# Autodesk Inventor assembly: Gondola
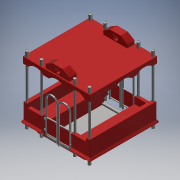
[picture p0: Inventor's stored thumbnail of the model, 180x180]
Saved by Autodesk Inventor 2018 (Build 220112000, 112)
## iProperties
Created: 2018-02-09
Part Number: Gondola
Document SubType Name: Assembly
Designer: Joey
Author: Joey
## Documents named in this file (13)
- M:\TPS\9th Grade\CADD 2017-2018\Current\Ferris Wheel Group Project\Group Project Week 3\Gondola\Gondola.iam
- M:\TPS\9th Grade\CADD 2017-2018\Current\Ferris Wheel Group Project\Group Project Week 3\Gondola\Gondola Body.ipt
- M:\TPS\9th Grade\CADD 2017-2018\Current\Ferris Wheel Group Project\Group Project Week 3\Gondola\Gondola Poles.ipt
- M:\TPS\9th Grade\CADD 2017-2018\Current\Ferris Wheel Group Project\Group Project Week 3\Gondola\Gondola Top Frame.ipt
- M:\TPS\9th Grade\CADD 2017-2018\Current\Ferris Wheel Group Project\Group Project Week 3\Gondola\Gondola Top.ipt
- M:\TPS\9th Grade\CADD 2017-2018\Current\Ferris Wheel Group Project\Group Project Week 3\Gondola\Gondola Pole Caps.ipt
- M:\TPS\9th Grade\CADD 2017-2018\Current\Ferris Wheel Group Project\Group Project Week 3\Gondola\Gondola Base Plate.ipt
- M:\TPS\9th Grade\CADD 2017-2018\Current\Ferris Wheel Group Project\Group Project Week 3\Gondola\Door Hinge.ipt
- M:\TPS\9th Grade\CADD 2017-2018\Current\Ferris Wheel Group Project\Group Project Week 3\Gondola\Door Hinge Pin.ipt
- M:\TPS\9th Grade\CADD 2017-2018\Current\Ferris Wheel Group Project\Group Project Week 3\Gondola\Left Door.iam
- M:\TPS\9th Grade\CADD 2017-2018\Current\Ferris Wheel Group Project\Group Project Week 3\Gondola\Hinge Pin Nut.ipt
- M:\TPS\9th Grade\CADD 2017-2018\Current\Ferris Wheel Group Project\Group Project Week 3\Gondola\Hinge Pin.ipt
- M:\TPS\9th Grade\CADD 2017-2018\Current\Ferris Wheel Group Project\Group Project Week 3\Gondola\Right Door.iam
## Components (65 placed, 12 different names)
1. Gondola Body:1 — Mate:1, Mate:2, Flush:1, Mate:8, Mate:9, Mate:10, Mate:11, Mate:12, Mate:13, Mate:14, Mate:15, Mate:16, Mate:17, Mate:18, Mate:19, Mate:20, Mate:21, Mate:22, Mate:23, Mate:24, Mate:25, Mate:26, Mate:27, Mate:28, Mate:29, Mate:30, Mate:31, Mate:32, Mate:33, Mate:34
2. Gondola Poles:1 — Mate:1, Mate:2, Flush:1, Mate:6, Mate:7, Flush:2, Insert:1, Insert:2, Insert:3, Insert:4, Insert:5, Insert:6, Insert:7, Insert:8, Insert:9, Insert:10, Insert:11, Insert:12, Insert:13, Insert:14, Insert:15, Insert:16
3. Gondola Top Frame:1 — Mate:3, Mate:4, Mate:5, Mate:6, Mate:7
4. Gondola Top:1 — Mate:3, Mate:4, Mate:5, Flush:2
5. Gondola Pole Caps:1 — Insert:9
6. Gondola Pole Caps:2 — Insert:10
7. Gondola Pole Caps:3 — Insert:11
8. Gondola Pole Caps:4 — Insert:12
9. Gondola Pole Caps:5 — Insert:16
10. Gondola Pole Caps:6 — Insert:15
11. Gondola Pole Caps:7 — Insert:14
12. Gondola Pole Caps:8 — Insert:13
13. Gondola Pole Caps:9 — Insert:5
14. Gondola Pole Caps:10 — Insert:6
15. Gondola Pole Caps:11 — Insert:7
16. Gondola Pole Caps:12 — Insert:8
17. Gondola Pole Caps:13 — Insert:1
18. Gondola Pole Caps:14 — Insert:2
19. Gondola Pole Caps:15 — Insert:3
20. Gondola Pole Caps:16 — Insert:4
21. Gondola Base Plate:1 — Mate:8, Mate:9, Mate:10
22. Door Hinge:1 — Mate:14, Mate:15, Mate:16, Insert:31, Insert:32
23. Door Hinge:2 — Mate:11, Mate:12, Mate:13, Insert:29, Insert:30, Mate:35, Mate:36
24. Door Hinge:3 — Mate:17, Mate:18, Mate:19, Insert:25, Insert:26, Mate:37, Mate:38
25. Door Hinge:4 — Mate:20, Mate:21, Mate:22, Insert:27, Insert:28
26. Door Hinge:5 — Mate:29, Mate:30, Mate:31, Insert:19, Insert:20
27. Door Hinge:6 — Mate:32, Mate:33, Mate:34, Insert:17, Insert:18, Mate:39, Mate:40
28. Door Hinge:7 — Mate:26, Mate:27, Mate:28, Insert:21, Insert:22
29. Door Hinge:8 — Mate:23, Mate:24, Mate:25, Insert:23, Insert:24, Mate:41, Mate:42
30. Door Hinge Pin:1 — Insert:18
31. Door Hinge Pin:2 — Insert:20
32. Door Hinge Pin:3 — Insert:17
33. Door Hinge Pin:4 — Insert:19
34. Door Hinge Pin:5 — Insert:32
35. Door Hinge Pin:6 — Insert:31
36. Door Hinge Pin:7 — Insert:30
37. Door Hinge Pin:8 — Insert:29
38. Door Hinge Pin:9 — Insert:25
39. Door Hinge Pin:10 — Insert:26
40. Door Hinge Pin:11 — Insert:27
41. Door Hinge Pin:12 — Insert:28
42. Door Hinge Pin:13 — Insert:21
43. Door Hinge Pin:14 — Insert:24
44. Door Hinge Pin:15 — Insert:23
45. Door Hinge Pin:16 — Insert:22
46. Left Door:1 [sub-assembly] — Mate:35, Mate:36, Insert:33, Insert:35, Insert:36, Insert:37
47. Hinge Pin Nut:1 — Insert:35
48. Hinge Pin:1 — Insert:37
49. Hinge Pin Nut:2 — Insert:36
50. Hinge Pin:2 — Insert:33
51. Right Door:1 [sub-assembly] — Mate:37, Mate:38, Insert:38, Insert:39, Insert:40, Insert:41
52. Hinge Pin Nut:3 — Insert:40
53. Hinge Pin:3 — Insert:38
54. Hinge Pin Nut:4 — Insert:41
55. Hinge Pin:4 — Insert:39
56. Left Door:2 [sub-assembly] — Mate:41, Mate:42, Insert:46, Insert:47, Insert:48, Insert:49
57. Right Door:2 [sub-assembly] — Mate:39, Mate:40, Insert:42, Insert:43, Insert:44, Insert:45
58. Hinge Pin Nut:5 — Insert:44
59. Hinge Pin:5 — Insert:42
60. Hinge Pin Nut:6 — Insert:45
61. Hinge Pin:6 — Insert:43
62. Hinge Pin Nut:7 — Insert:49
63. Hinge Pin:7 — Insert:47
64. Hinge Pin Nut:8 — Insert:48
65. Hinge Pin:8 — Insert:46
## Relationships (92: Insert 48, Mate 42, Flush 2)
- Mate:1: Gondola Body:1 ↔ Gondola Poles:1
- Mate:2: Gondola Body:1 ↔ Gondola Poles:1
- Flush:1 (-152.4 mm): Gondola Body:1 ↔ Gondola Poles:1
- Mate:3: Gondola Top Frame:1 ↔ Gondola Top:1
- Mate:4: Gondola Top Frame:1 ↔ Gondola Top:1
- Mate:5: Gondola Top Frame:1 ↔ Gondola Top:1
- Mate:6: Gondola Poles:1 ↔ Gondola Top Frame:1
- Mate:7: Gondola Poles:1 ↔ Gondola Top Frame:1
- Flush:2 (152.4 mm): Gondola Poles:1 ↔ Gondola Top:1
- Insert:1: Gondola Poles:1 ↔ Gondola Pole Caps:13
- Insert:2: Gondola Poles:1 ↔ Gondola Pole Caps:14
- Insert:3: Gondola Poles:1 ↔ Gondola Pole Caps:15
- Insert:4: Gondola Poles:1 ↔ Gondola Pole Caps:16
- Insert:5: Gondola Poles:1 ↔ Gondola Pole Caps:9
- Insert:6: Gondola Poles:1 ↔ Gondola Pole Caps:10
- Insert:7: Gondola Poles:1 ↔ Gondola Pole Caps:11
- Insert:8: Gondola Poles:1 ↔ Gondola Pole Caps:12
- Insert:9: Gondola Poles:1 ↔ Gondola Pole Caps:1
- Insert:10: Gondola Poles:1 ↔ Gondola Pole Caps:2
- Insert:11: Gondola Poles:1 ↔ Gondola Pole Caps:3
- Insert:12: Gondola Poles:1 ↔ Gondola Pole Caps:4
- Insert:13: Gondola Poles:1 ↔ Gondola Pole Caps:8
- Insert:14: Gondola Poles:1 ↔ Gondola Pole Caps:7
- Insert:15: Gondola Poles:1 ↔ Gondola Pole Caps:6
- Insert:16: Gondola Poles:1 ↔ Gondola Pole Caps:5
- Mate:8: Gondola Body:1 ↔ Gondola Base Plate:1
- Mate:9: Gondola Body:1 ↔ Gondola Base Plate:1
- Mate:10: Gondola Body:1 ↔ Gondola Base Plate:1
- Mate:11: Gondola Body:1 ↔ Door Hinge:2
- Mate:12: Gondola Body:1 ↔ Door Hinge:2
- Mate:13: Gondola Body:1 ↔ Door Hinge:2
- Mate:14: Gondola Body:1 ↔ Door Hinge:1
- Mate:15: Gondola Body:1 ↔ Door Hinge:1
- Mate:16: Gondola Body:1 ↔ Door Hinge:1
- Mate:17: Gondola Body:1 ↔ Door Hinge:3
- Mate:18: Gondola Body:1 ↔ Door Hinge:3
- Mate:19: Gondola Body:1 ↔ Door Hinge:3
- Mate:20: Gondola Body:1 ↔ Door Hinge:4
- Mate:21: Gondola Body:1 ↔ Door Hinge:4
- Mate:22: Gondola Body:1 ↔ Door Hinge:4
- Mate:23: Gondola Body:1 ↔ Door Hinge:8
- Mate:24: Gondola Body:1 ↔ Door Hinge:8
- Mate:25: Gondola Body:1 ↔ Door Hinge:8
- Mate:26: Gondola Body:1 ↔ Door Hinge:7
- Mate:27: Gondola Body:1 ↔ Door Hinge:7
- Mate:28: Gondola Body:1 ↔ Door Hinge:7
- Mate:29: Gondola Body:1 ↔ Door Hinge:5
- Mate:30: Gondola Body:1 ↔ Door Hinge:5
- Mate:31: Gondola Body:1 ↔ Door Hinge:5
- Mate:32: Gondola Body:1 ↔ Door Hinge:6
- Mate:33: Gondola Body:1 ↔ Door Hinge:6
- Mate:34: Gondola Body:1 ↔ Door Hinge:6
- Insert:17: Door Hinge:6 ↔ Door Hinge Pin:3
- Insert:18: Door Hinge:6 ↔ Door Hinge Pin:1
- Insert:19: Door Hinge:5 ↔ Door Hinge Pin:4
- Insert:20: Door Hinge:5 ↔ Door Hinge Pin:2
- Insert:21: Door Hinge:7 ↔ Door Hinge Pin:13
- Insert:22: Door Hinge:7 ↔ Door Hinge Pin:16
- Insert:23: Door Hinge:8 ↔ Door Hinge Pin:15
- Insert:24: Door Hinge:8 ↔ Door Hinge Pin:14
- Insert:25: Door Hinge:3 ↔ Door Hinge Pin:9
- Insert:26: Door Hinge:3 ↔ Door Hinge Pin:10
- Insert:27: Door Hinge:4 ↔ Door Hinge Pin:11
- Insert:28: Door Hinge:4 ↔ Door Hinge Pin:12
- Insert:29: Door Hinge:2 ↔ Door Hinge Pin:8
- Insert:30: Door Hinge:2 ↔ Door Hinge Pin:7
- Insert:31: Door Hinge:1 ↔ Door Hinge Pin:6
- Insert:32: Door Hinge:1 ↔ Door Hinge Pin:5
- Mate:35: Door Hinge:2 ↔ Left Door:1
- Mate:36: Door Hinge:2 ↔ Left Door:1
- Insert:33: Left Door:1 ↔ Hinge Pin:2
- Insert:35: Left Door:1 ↔ Hinge Pin Nut:1
- Insert:36: Left Door:1 ↔ Hinge Pin Nut:2
- Insert:37: Left Door:1 ↔ Hinge Pin:1
- Mate:37: Door Hinge:3 ↔ Right Door:1
- Mate:38: Door Hinge:3 ↔ Right Door:1
- Insert:38: Right Door:1 ↔ Hinge Pin:3
- Insert:39: Right Door:1 ↔ Hinge Pin:4
- Insert:40: Right Door:1 ↔ Hinge Pin Nut:3
- Insert:41: Right Door:1 ↔ Hinge Pin Nut:4
- Mate:39: Door Hinge:6 ↔ Right Door:2
- Mate:40: Door Hinge:6 ↔ Right Door:2
- Mate:41: Door Hinge:8 ↔ Left Door:2
- Mate:42: Door Hinge:8 ↔ Left Door:2
- Insert:42: Right Door:2 ↔ Hinge Pin:5
- Insert:43: Right Door:2 ↔ Hinge Pin:6
- Insert:44: Right Door:2 ↔ Hinge Pin Nut:5
- Insert:45: Right Door:2 ↔ Hinge Pin Nut:6
- Insert:46: Left Door:2 ↔ Hinge Pin:8
- Insert:47: Left Door:2 ↔ Hinge Pin:7
- Insert:48: Left Door:2 ↔ Hinge Pin Nut:8
- Insert:49: Left Door:2 ↔ Hinge Pin Nut:7
